# Autodesk Inventor assembly: 110033226_iam_04_大橋塔樓
(part 2 of 2)
981. 110033226_ipt_10_木板條:51
982. 110033226_ipt_10_木板條:52
983. 110033226_ipt_10_木板條:53
984. 110033226_ipt_10_木板條:54
985. 110033226_ipt_10_木板條:55
986. 110033226_ipt_10_木板條:56
987. 110033226_ipt_10_木板條:57
988. 110033226_ipt_10_木板條:58
989. 110033226_ipt_10_木板條:59
990. 110033226_ipt_10_木板條:60
991. 110033226_ipt_10_木板條:61
992. 110033226_ipt_10_木板條:62
993. 110033226_ipt_10_木板條:63
994. 110033226_ipt_10_木板條:64
995. 110033226_ipt_10_木板條:65
996. 110033226_ipt_10_木板條:66
997. 110033226_ipt_10_木板條:67
998. 110033226_ipt_10_木板條:68
999. 110033226_ipt_10_木板條:69
1000. 110033226_ipt_10_木板條:70
1001. 110033226_ipt_10_木板條:71
1002. 110033226_ipt_10_木板條:72
1003. 110033226_ipt_10_木板條:73
1004. 110033226_ipt_10_木板條:74
1005. 110033226_ipt_10_木板條:75
1006. 110033226_ipt_22_塔樓牆壁:238 — 貼合:219, 貼合:220, 貼合:221
1007. 110033226_ipt_22_塔樓牆壁:241
1008. 110033226_ipt_22_塔樓牆壁:242
1009. 110033226_ipt_22_塔樓牆壁:243
1010. 110033226_ipt_22_塔樓牆壁:236 — 貼合:222, 貼合:223, 貼合:224
1011. 110033226_ipt_22_塔樓牆壁:244
1012. 110033226_ipt_22_塔樓牆壁:245
1013. 110033226_ipt_22_塔樓牆壁:240 — 貼合:225, 貼合:226, 貼合:227
1014. 110033226_ipt_22_塔樓牆壁:246
1015. 110033226_ipt_22_塔樓牆壁:247
1016. 110033226_ipt_22_塔樓牆壁:248 — 貼合:228, 貼合:229, 貼合:230
1017. 110033226_ipt_22_塔樓牆壁:249
1018. 110033226_ipt_22_塔樓牆壁:250
1019. 110033226_ipt_22_塔樓牆壁:251
1020. 110033226_ipt_22_塔樓牆壁:252
1021. 110033226_ipt_22_塔樓牆壁:253
1022. 110033226_ipt_22_塔樓牆壁:254
1023. 110033226_ipt_22_塔樓牆壁:255
1024. 110033226_ipt_22_塔樓牆壁:256
1025. 110033226_ipt_22_塔樓牆壁:257
1026. 110033226_ipt_22_塔樓牆壁:258
1027. 110033226_ipt_22_塔樓牆壁:259
1028. 110033226_ipt_22_塔樓牆壁:260
1029. 110033226_ipt_22_塔樓牆壁:261 — 貼合:239
1030. 110033226_ipt_22_塔樓牆壁:262
1031. 110033226_ipt_22_塔樓牆壁:263
1032. 110033226_ipt_22_塔樓牆壁:264
1033. 110033226_ipt_22_塔樓牆壁:265
1034. 110033226_ipt_22_塔樓牆壁:266
1035. 110033226_ipt_22_塔樓牆壁:267
1036. 110033226_ipt_22_塔樓牆壁:268
1037. 110033226_ipt_22_塔樓牆壁:269
1038. 110033226_ipt_22_塔樓牆壁:270
1039. 110033226_ipt_22_塔樓牆壁:271
1040. 110033226_ipt_22_塔樓牆壁:272
1041. 110033226_ipt_22_塔樓牆壁:273 — 貼合:237, 貼合:238
1042. 110033226_ipt_22_塔樓牆壁:274
1043. 110033226_ipt_22_塔樓牆壁:275
1044. 110033226_ipt_22_塔樓牆壁:276
1045. 110033226_ipt_22_塔樓牆壁:277
1046. 110033226_ipt_22_塔樓牆壁:278
1047. 110033226_ipt_22_塔樓牆壁:279
1048. 110033226_ipt_22_塔樓牆壁:280
1049. 110033226_ipt_22_塔樓牆壁:281
1050. 110033226_ipt_22_塔樓牆壁:282
1051. 110033226_ipt_22_塔樓牆壁:283
1052. 110033226_ipt_22_塔樓牆壁:284
1053. 110033226_ipt_22_塔樓牆壁:285
1054. 110033226_ipt_22_塔樓牆壁:286
1055. 110033226_ipt_22_塔樓牆壁:287
1056. 110033226_ipt_22_塔樓牆壁:288
1057. 110033226_ipt_22_塔樓牆壁:289 — 貼合:234, 貼合:235, 貼合:236
1058. 110033226_ipt_22_塔樓牆壁:290
1059. 110033226_ipt_22_塔樓牆壁:291
1060. 110033226_ipt_22_塔樓牆壁:292
1061. 110033226_ipt_22_塔樓牆壁:293
1062. 110033226_ipt_22_塔樓牆壁:294
1063. 110033226_ipt_22_塔樓牆壁:295
1064. 110033226_ipt_22_塔樓牆壁:296
1065. 110033226_ipt_22_塔樓牆壁:297
1066. 110033226_ipt_23_塔樓門口:2 — 貼合:154, 貼合:155, 貼合:156, 貼合:160, 貼合:161, 貼合:162, 貼合:188, 貼合:189
1067. 110033226_ipt_23_塔樓門口:3 — 貼合:187
1068. 110033226_ipt_23_塔樓門口:5
1069. 110033226_ipt_23_塔樓門口:6
1070. 110033226_ipt_23_塔樓門口:7
1071. 110033226_ipt_23_塔樓門口:8
1072. 110033226_ipt_07_磚塊樺木(2x1):229 — 貼合:50, 貼合:51, 貼合:53, 貼合:54, 貼合:56
1073. 110033226_ipt_06_磚塊樺木(1x1):227 — 貼合:54, 貼合:55, 貼合:56
1074. 110033226_ipt_07_磚塊樺木(2x1):230
1075. 110033226_ipt_06_磚塊樺木(1x1):230
1076. 110033226_ipt_07_磚塊樺木(2x1):232 — 貼合:163, 貼合:164
1077. 110033226_ipt_06_磚塊樺木(1x1):232
1078. 110033226_ipt_07_磚塊樺木(2x1):233
1079. 110033226_ipt_06_磚塊樺木(1x1):233 — 貼合:169
1080. 110033226_ipt_07_磚塊樺木(2x1):255
1081. 110033226_ipt_06_磚塊樺木(1x1):255
1082. 110033226_ipt_07_磚塊樺木(2x1):256
1083. 110033226_ipt_06_磚塊樺木(1x1):256
1084. 110033226_ipt_07_磚塊樺木(2x1):257
1085. 110033226_ipt_06_磚塊樺木(1x1):257
1086. 110033226_ipt_07_磚塊樺木(2x1):258
1087. 110033226_ipt_06_磚塊樺木(1x1):258
1088. 110033226_ipt_07_磚塊樺木(2x1):260
1089. 110033226_ipt_06_磚塊樺木(1x1):260
1090. 110033226_ipt_07_磚塊樺木(2x1):261
1091. 110033226_ipt_06_磚塊樺木(1x1):261
1092. 110033226_ipt_07_磚塊樺木(2x1):262
1093. 110033226_ipt_06_磚塊樺木(1x1):262
1094. 110033226_ipt_07_磚塊樺木(2x1):263
1095. 110033226_ipt_06_磚塊樺木(1x1):263
1096. 110033226_ipt_07_磚塊樺木(2x1):265
1097. 110033226_ipt_06_磚塊樺木(1x1):265
1098. 110033226_ipt_07_磚塊樺木(2x1):266
1099. 110033226_ipt_06_磚塊樺木(1x1):266
1100. 110033226_ipt_07_磚塊樺木(2x1):267
1101. 110033226_ipt_06_磚塊樺木(1x1):267
1102. 110033226_ipt_07_磚塊樺木(2x1):268
1103. 110033226_ipt_06_磚塊樺木(1x1):268
1104. 110033226_ipt_07_磚塊樺木(2x1):270
1105. 110033226_ipt_06_磚塊樺木(1x1):270
1106. 110033226_ipt_07_磚塊樺木(2x1):271
1107. 110033226_ipt_06_磚塊樺木(1x1):271
1108. 110033226_ipt_07_磚塊樺木(2x1):272
1109. 110033226_ipt_06_磚塊樺木(1x1):272
1110. 110033226_ipt_07_磚塊樺木(2x1):273
1111. 110033226_ipt_06_磚塊樺木(1x1):273
1112. 110033226_ipt_07_磚塊樺木(2x1):275
1113. 110033226_ipt_06_磚塊樺木(1x1):275
1114. 110033226_ipt_07_磚塊樺木(2x1):276
1115. 110033226_ipt_06_磚塊樺木(1x1):276
1116. 110033226_ipt_07_磚塊樺木(2x1):277
1117. 110033226_ipt_06_磚塊樺木(1x1):277
1118. 110033226_ipt_07_磚塊樺木(2x1):278
1119. 110033226_ipt_06_磚塊樺木(1x1):278
1120. 110033226_ipt_07_磚塊樺木(2x1):280
1121. 110033226_ipt_06_磚塊樺木(1x1):280
1122. 110033226_ipt_07_磚塊樺木(2x1):281
1123. 110033226_ipt_06_磚塊樺木(1x1):281
1124. 110033226_ipt_07_磚塊樺木(2x1):282
1125. 110033226_ipt_06_磚塊樺木(1x1):282
1126. 110033226_ipt_07_磚塊樺木(2x1):283
1127. 110033226_ipt_06_磚塊樺木(1x1):283
1128. 110033226_ipt_07_磚塊樺木(2x1):285
1129. 110033226_ipt_06_磚塊樺木(1x1):285
1130. 110033226_ipt_07_磚塊樺木(2x1):286
1131. 110033226_ipt_06_磚塊樺木(1x1):286
1132. 110033226_ipt_07_磚塊樺木(2x1):287
1133. 110033226_ipt_06_磚塊樺木(1x1):287
1134. 110033226_ipt_07_磚塊樺木(2x1):288
1135. 110033226_ipt_06_磚塊樺木(1x1):288
1136. 110033226_ipt_07_磚塊樺木(2x1):290
1137. 110033226_ipt_06_磚塊樺木(1x1):290
1138. 110033226_ipt_07_磚塊樺木(2x1):291
1139. 110033226_ipt_06_磚塊樺木(1x1):291
1140. 110033226_ipt_07_磚塊樺木(2x1):292
1141. 110033226_ipt_06_磚塊樺木(1x1):292
1142. 110033226_ipt_07_磚塊樺木(2x1):293
1143. 110033226_ipt_06_磚塊樺木(1x1):293
1144. 110033226_ipt_07_磚塊樺木(2x1):295
1145. 110033226_ipt_06_磚塊樺木(1x1):295
1146. 110033226_ipt_07_磚塊樺木(2x1):296
1147. 110033226_ipt_06_磚塊樺木(1x1):296
1148. 110033226_ipt_07_磚塊樺木(2x1):297
1149. 110033226_ipt_06_磚塊樺木(1x1):297
1150. 110033226_ipt_07_磚塊樺木(2x1):298 — 貼合:240
1151. 110033226_ipt_06_磚塊樺木(1x1):298
## Component patterns: (2 elements), (2 elements), (2 elements, first: 110033226_ipt_16_圍牆:1), (12 elements), (2 elements), (14 elements, first: 110033226_ipt_21_柵欄:1), (10 elements, first: 110033226_ipt_21_柵欄:2), (4 elements), (3 elements), (25 elements, first: 110033226_ipt_22_塔樓牆壁:2), (10 elements, first: 110033226_ipt_22_塔樓牆壁:46), (6 elements, first: 110033226_ipt_11_樓梯支架:41), (3 elements, first: 110033226_ipt_10_木板條:3), (6 elements, first: 110033226_ipt_11_樓梯支架:40), (2 elements, first: 110033226_ipt_10_木板條:39), (3 elements), (7 elements, first: 110033226_ipt_22_塔樓牆壁:55), (2 elements, first: 110033226_ipt_22_塔樓牆壁:147), (14 elements, first: 110033226_ipt_22_塔樓牆壁:148), (5 elements), (2 elements), (20 elements, first: 110033226_ipt_07_磚塊樺木(2x1):234 + 110033226_ipt_06_磚塊樺木(1x1):234), (10 elements, first: 110033226_ipt_07_磚塊樺木(2x1):228 + 110033226_ipt_06_磚塊樺木(1x1):229), (10 elements, first: 110033226_ipt_06_磚塊樺木(1x1):299), (4 elements, first: 110033226_ipt_24_直條(3x1):1), (5 elements, first: 110033226_ipt_22_塔樓牆壁:194), (3 elements, first: 110033226_ipt_24_直條(3x1):5), (2 elements), (6 elements, first: 110033226_ipt_22_塔樓牆壁:193), (8 elements, first: 110033226_ipt_22_塔樓牆壁:217), (2 elements, first: 110033226_ipt_22_塔樓牆壁:225), (14 elements, first: 110033226_ipt_21_柵欄:26), (30 elements, first: 110033226_ipt_08_平滑面(3x1):67), (8 elements, first: 110033226_ipt_22_塔樓牆壁:227), (2 elements, first: 110033226_ipt_08_平滑面(3x1):100), (6 elements, first: 110033226_ipt_08_平滑面(3x1):101), (2 elements, first: 110033226_ipt_12_平滑面(2x1):1), (12 elements, first: 110033226_ipt_21_柵欄:42), (3 elements, first: 110033226_ipt_18_大橋圍牆:2), (3 elements, first: 110033226_ipt_18_大橋圍牆:1), (5 elements), (28 elements, first: 110033226_ipt_12_平滑面(2x1):4), (3 elements, first: 110033226_ipt_22_塔樓牆壁:298), (3 elements), (14 elements, first: 110033226_ipt_12_平滑面(2x1):35), (4 elements, first: 110033226_ipt_08_平滑面(3x1):110), (12 elements, first: 110033226_ipt_08_平滑面(3x1):108), (28 elements, first: 110033226_ipt_06_磚塊樺木(1x1):2 + 110033226_ipt_07_磚塊樺木(2x1):2 + 110033226_ipt_06_磚塊樺木(1x1):1 + 110033226_ipt_07_磚塊樺木(2x1):5), 元件陣列 2:2 (28 elements), (28 elements, first: 110033226_ipt_07_磚塊樺木(2x1):3 + 110033226_ipt_06_磚塊樺木(1x1):4 + 110033226_ipt_07_磚塊樺木(2x1):6 + 110033226_ipt_06_磚塊樺木(1x1):5), 元件陣列 1:2 (28 elements), (4 elements, first: 110033226_ipt_08_平滑面(3x1):1), 元件陣列 6:2 (4 elements), 元件陣列 6:3 (4 elements), 元件陣列 6:4 (4 elements), 元件陣列 6:5 (4 elements), 元件陣列 6:6 (4 elements), 元件陣列 6:7 (4 elements), 元件陣列 6:8 (4 elements), 元件陣列 6:9 (4 elements), 元件陣列 6:10 (4 elements), 元件陣列 6:11 (4 elements), 元件陣列 6:12 (4 elements), (4 elements, first: 110033226_ipt_08_平滑面(3x1):2), 元件陣列 8:2 (4 elements), (4 elements, first: 110033226_ipt_11_樓梯支架:1 + 110033226_ipt_11_樓梯支架:2), 元件陣列 17:2 (4 elements), 元件陣列 17:3 (4 elements), 元件陣列 17:4 (4 elements), (6 elements, first: 110033226_ipt_22_塔樓牆壁:1), 元件陣列 19:2 (6 elements), 元件陣列 19:3 (6 elements), (12 elements, first: 110033226_ipt_22_塔樓牆壁:104), 元件陣列 29:2 (12 elements), 元件陣列 29:3 (12 elements), (6 elements, first: 110033226_ipt_22_塔樓牆壁:146), 元件陣列 35:2 (6 elements), 元件陣列 35:3 (6 elements), 元件陣列 35:4 (6 elements), 元件陣列 35:5 (6 elements), (6 elements, first: 110033226_ipt_22_塔樓牆壁:192), 元件陣列 37:2 (6 elements), (2 elements), 元件陣列 14:2 (2 elements), 元件陣列 14:3 (2 elements), 元件陣列 14:4 (2 elements), 元件陣列 14:5 (2 elements), 元件陣列 14:6 (2 elements), 元件陣列 14:7 (2 elements), 元件陣列 14:8 (2 elements), 元件陣列 14:9 (2 elements), 元件陣列 14:10 (2 elements), (30 elements, first: 110033226_ipt_10_木板條:2), 元件陣列 23:2 (30 elements), (4 elements, first: 110033226_ipt_22_塔樓牆壁:238), (3 elements, first: 110033226_ipt_22_塔樓牆壁:236), (3 elements, first: 110033226_ipt_22_塔樓牆壁:240), (2 elements, first: 110033226_ipt_22_塔樓牆壁:248), 元件陣列 59:2 (4 elements), 元件陣列 60:2 (3 elements), 元件陣列 61:2 (3 elements), 元件陣列 62:2 (2 elements), 元件陣列 59:3 (4 elements), 元件陣列 60:3 (3 elements), 元件陣列 61:3 (3 elements), 元件陣列 62:3 (2 elements), 元件陣列 59:4 (4 elements), 元件陣列 60:4 (3 elements), 元件陣列 61:4 (3 elements), 元件陣列 62:4 (2 elements), 元件陣列 59:5 (4 elements), 元件陣列 60:5 (3 elements), 元件陣列 61:5 (3 elements), 元件陣列 62:5 (2 elements), (2 elements, first: 110033226_ipt_23_塔樓門口:2), 元件陣列 34:2 (2 elements), 元件陣列 34:3 (2 elements), (2 elements, first: 110033226_ipt_07_磚塊樺木(2x1):229 + 110033226_ipt_06_磚塊樺木(1x1):227), 元件陣列 12:2 (2 elements), 元件陣列 12:3 (2 elements), 元件陣列 12:4 (2 elements), 元件陣列 12:5 (2 elements), 元件陣列 12:6 (2 elements), 元件陣列 12:7 (2 elements), 元件陣列 12:8 (2 elements), 元件陣列 12:9 (2 elements), 元件陣列 12:10 (2 elements), 元件陣列 12:11 (2 elements), 元件陣列 12:12 (2 elements), 元件陣列 12:13 (2 elements), 元件陣列 12:14 (2 elements), 元件陣列 12:15 (2 elements), 元件陣列 12:16 (2 elements), 元件陣列 12:17 (2 elements), 元件陣列 12:18 (2 elements), 元件陣列 12:19 (2 elements), 元件陣列 12:20 (2 elements)
## Relationships (245: Mate 241, Symmetry 4)
- 貼合:1 [Mate]: 110033226_ipt_05_房子底座:1 ↔ 110033226_ipt_07_磚塊樺木(2x1):6
- 貼合:2 [Mate]: 110033226_ipt_05_房子底座:1 ↔ 110033226_ipt_07_磚塊樺木(2x1):6
- 貼合:3 [Mate]: 110033226_ipt_05_房子底座:1 ↔ 110033226_ipt_07_磚塊樺木(2x1):6
- 貼合:4 [Mate]: 110033226_ipt_05_房子底座:1 ↔ 110033226_ipt_06_磚塊樺木(1x1):5
- 貼合:5 [Mate]: 110033226_ipt_05_房子底座:1 ↔ 110033226_ipt_06_磚塊樺木(1x1):5
- 貼合:6 [Mate]: 110033226_ipt_07_磚塊樺木(2x1):6 ↔ 110033226_ipt_06_磚塊樺木(1x1):5
- 貼合:7 [Mate]: 110033226_ipt_07_磚塊樺木(2x1):3 ↔ 110033226_ipt_07_磚塊樺木(2x1):6
- 貼合:8 [Mate]: 110033226_ipt_07_磚塊樺木(2x1):3 ↔ 110033226_ipt_07_磚塊樺木(2x1):6
- 貼合:9 [Mate]: 110033226_ipt_07_磚塊樺木(2x1):3 ↔ 110033226_ipt_06_磚塊樺木(1x1):5
- 貼合:10 [Mate]: 110033226_ipt_06_磚塊樺木(1x1):4 ↔ 110033226_ipt_07_磚塊樺木(2x1):6
- 貼合:11 [Mate]: 110033226_ipt_06_磚塊樺木(1x1):4 ↔ 110033226_ipt_07_磚塊樺木(2x1):6
- 貼合:12 [Mate]: 110033226_ipt_07_磚塊樺木(2x1):3 ↔ 110033226_ipt_06_磚塊樺木(1x1):4
- 貼合:13 [Mate]: 110033226_ipt_05_房子底座:1 ↔ 110033226_ipt_07_磚塊樺木(2x1):5
- 貼合:14 [Mate]: 110033226_ipt_05_房子底座:1 ↔ 110033226_ipt_07_磚塊樺木(2x1):5
- 貼合:15 [Mate]: 110033226_ipt_05_房子底座:1 ↔ 110033226_ipt_07_磚塊樺木(2x1):5
- 貼合:16 [Mate]: 110033226_ipt_05_房子底座:1 ↔ 110033226_ipt_06_磚塊樺木(1x1):1
- 貼合:17 [Mate]: 110033226_ipt_05_房子底座:1 ↔ 110033226_ipt_06_磚塊樺木(1x1):1
- 貼合:18 [Mate]: 110033226_ipt_06_磚塊樺木(1x1):1 ↔ 110033226_ipt_07_磚塊樺木(2x1):5
- 貼合:19 [Mate]: 110033226_ipt_07_磚塊樺木(2x1):2 ↔ 110033226_ipt_06_磚塊樺木(1x1):1
- 貼合:20 [Mate]: 110033226_ipt_07_磚塊樺木(2x1):2 ↔ 110033226_ipt_07_磚塊樺木(2x1):5
- 貼合:21 [Mate]: 110033226_ipt_07_磚塊樺木(2x1):2 ↔ 110033226_ipt_06_磚塊樺木(1x1):1
- 貼合:22 [Mate]: 110033226_ipt_06_磚塊樺木(1x1):2 ↔ 110033226_ipt_07_磚塊樺木(2x1):5
- 貼合:23 [Mate]: 110033226_ipt_06_磚塊樺木(1x1):2 ↔ 110033226_ipt_07_磚塊樺木(2x1):2
- 貼合:24 [Mate]: 110033226_ipt_06_磚塊樺木(1x1):2 ↔ 110033226_ipt_07_磚塊樺木(2x1):5
- 貼合:25 [Mate]: 110033226_ipt_16_圍牆:1 ↔ 110033226_ipt_07_磚塊樺木(2x1):172
- 貼合:26 [Mate]: 110033226_ipt_16_圍牆:1 ↔ 110033226_ipt_07_磚塊樺木(2x1):172
- 貼合:27 [Mate]: 110033226_ipt_16_圍牆:1 ↔ 110033226_ipt_07_磚塊樺木(2x1):172
- 貼合:28 [Mate]: 110033226_ipt_07_磚塊樺木(2x1):1 ↔ 110033226_ipt_07_磚塊樺木(2x1):214
- 貼合:29 [Mate]: 110033226_ipt_07_磚塊樺木(2x1):1 ↔ 110033226_ipt_07_磚塊樺木(2x1):214
- 貼合:30 [Mate]: 110033226_ipt_07_磚塊樺木(2x1):1 ↔ 110033226_ipt_06_磚塊樺木(1x1):213
- 貼合:31 [Mate]: 110033226_ipt_07_磚塊樺木(2x1):165 ↔ 110033226_ipt_08_平滑面(3x1):1
- 貼合:32 [Mate]: 110033226_ipt_07_磚塊樺木(2x1):59 ↔ 110033226_ipt_08_平滑面(3x1):1
- 貼合:33 [Mate]: 110033226_ipt_07_磚塊樺木(2x1):163 ↔ 110033226_ipt_08_平滑面(3x1):1
- 貼合:34 [Mate]: 110033226_ipt_07_磚塊樺木(2x1):225 ↔ 110033226_ipt_08_平滑面(3x1):2
- 貼合:35 [Mate]: 110033226_ipt_07_磚塊樺木(2x1):169 ↔ 110033226_ipt_08_平滑面(3x1):2
- 貼合:36 [Mate]: 110033226_ipt_06_磚塊樺木(1x1):224 ↔ 110033226_ipt_08_平滑面(3x1):2
- 貼合:37 [Mate]: 110033226_ipt_20_塔樓窗戶:1 ↔ 110033226_ipt_07_磚塊樺木(2x1):21
- 貼合:38 [Mate]: 110033226_ipt_20_塔樓窗戶:1 ↔ 110033226_ipt_06_磚塊樺木(1x1):50
- 貼合:39 [Mate]: 110033226_ipt_20_塔樓窗戶:1 ↔ 110033226_ipt_07_磚塊樺木(2x1):52
- 貼合:40 [Mate]: 110033226_ipt_20_塔樓窗戶:1 ↔ 110033226_ipt_07_磚塊樺木(2x1):21
- 貼合:41 [Mate]: 110033226_ipt_20_塔樓窗戶:2 ↔ 110033226_ipt_07_磚塊樺木(2x1):201
- 貼合:42 [Mate]: 110033226_ipt_20_塔樓窗戶:2 ↔ 110033226_ipt_06_磚塊樺木(1x1):175
- 貼合:43 [Mate]: 110033226_ipt_20_塔樓窗戶:2 ↔ 110033226_ipt_07_磚塊樺木(2x1):201
- 貼合:44 [Mate]: 110033226_ipt_21_柵欄:1 ↔ 110033226_ipt_08_平滑面(3x1):13
- 貼合:45 [Mate]: 110033226_ipt_21_柵欄:1 ↔ 110033226_ipt_08_平滑面(3x1):13
- 貼合:46 [Mate]: 110033226_ipt_21_柵欄:1 ↔ 110033226_ipt_08_平滑面(3x1):13
- 貼合:47 [Mate]: 110033226_ipt_21_柵欄:2 ↔ 110033226_ipt_08_平滑面(3x1):13
- 貼合:48 [Mate]: 110033226_ipt_21_柵欄:1 ↔ 110033226_ipt_21_柵欄:2
- 貼合:49 [Mate]: 110033226_ipt_21_柵欄:2 ↔ 110033226_ipt_08_平滑面(3x1):12
- 貼合:50 [Mate]: 110033226_ipt_08_平滑面(3x1):48 ↔ 110033226_ipt_07_磚塊樺木(2x1):229
- 貼合:51 [Mate]: 110033226_ipt_08_平滑面(3x1):48 ↔ 110033226_ipt_07_磚塊樺木(2x1):229
- 貼合:53 [Mate]: 110033226_ipt_08_平滑面(3x1):48 ↔ 110033226_ipt_07_磚塊樺木(2x1):229
- 貼合:54 [Mate]: 110033226_ipt_07_磚塊樺木(2x1):229 ↔ 110033226_ipt_06_磚塊樺木(1x1):227
- 貼合:55 [Mate]: 110033226_ipt_08_平滑面(3x1):48 ↔ 110033226_ipt_06_磚塊樺木(1x1):227
- 貼合:56 [Mate]: 110033226_ipt_07_磚塊樺木(2x1):229 ↔ 110033226_ipt_06_磚塊樺木(1x1):227
- 貼合:57 [Mate]: 110033226_ipt_07_磚塊樺木(2x1):228 ↔ 110033226_ipt_08_平滑面(3x1):43
- 貼合:58 [Mate]: 110033226_ipt_07_磚塊樺木(2x1):228 ↔ 110033226_ipt_08_平滑面(3x1):43
- 貼合:59 [Mate]: 110033226_ipt_07_磚塊樺木(2x1):228 ↔ 110033226_ipt_08_平滑面(3x1):39
- 貼合:60 [Mate]: 110033226_ipt_06_磚塊樺木(1x1):229 ↔ 110033226_ipt_08_平滑面(3x1):35
- 貼合:61 [Mate]: 110033226_ipt_07_磚塊樺木(2x1):228 ↔ 110033226_ipt_06_磚塊樺木(1x1):229
- 貼合:62 [Mate]: 110033226_ipt_07_磚塊樺木(2x1):228 ↔ 110033226_ipt_06_磚塊樺木(1x1):229
- 貼合:63 [Mate]: 110033226_ipt_08_平滑面(3x1):37 ↔ 110033226_ipt_11_樓梯支架:1
- 貼合:64 [Mate]: 110033226_ipt_08_平滑面(3x1):37 ↔ 110033226_ipt_11_樓梯支架:1
- 貼合:65 [Mate]: 110033226_ipt_08_平滑面(3x1):41 ↔ 110033226_ipt_11_樓梯支架:1
- 貼合:66 [Mate]: 110033226_ipt_11_樓梯支架:1 ↔ 110033226_ipt_11_樓梯支架:2
- 貼合:67 [Mate]: 110033226_ipt_11_樓梯支架:1 ↔ 110033226_ipt_11_樓梯支架:2
- 貼合:68 [Mate]: 110033226_ipt_11_樓梯支架:1 ↔ 110033226_ipt_11_樓梯支架:2
- 貼合:69 [Mate]: 110033226_ipt_08_平滑面(3x1):58 ↔ 110033226_ipt_11_樓梯支架:27
- 貼合:70 [Mate]: 110033226_ipt_08_平滑面(3x1):58 ↔ 110033226_ipt_11_樓梯支架:19
- 貼合:71 [Mate]: 110033226_ipt_08_平滑面(3x1):58 ↔ 110033226_ipt_11_樓梯支架:27
- 貼合:72 [Mate]: 110033226_ipt_08_平滑面(3x1):59 ↔ 110033226_ipt_11_樓梯支架:35
- 貼合:73 [Mate]: 110033226_ipt_08_平滑面(3x1):59 ↔ 110033226_ipt_11_樓梯支架:27
- 貼合:74 [Mate]: 110033226_ipt_08_平滑面(3x1):59 ↔ 110033226_ipt_11_樓梯支架:19
- 貼合:75 [Mate]: 110033226_ipt_08_平滑面(3x1):60 ↔ 110033226_ipt_11_樓梯支架:10
- 貼合:76 [Mate]: 110033226_ipt_08_平滑面(3x1):61 ↔ 110033226_ipt_11_樓梯支架:33
- 貼合:77 [Mate]: 110033226_ipt_08_平滑面(3x1):64 ↔ 110033226_ipt_11_樓梯支架:7
- 貼合:78 [Mate]: 110033226_ipt_08_平滑面(3x1):62 ↔ 110033226_ipt_11_樓梯支架:8
- 貼合:79 [Mate]: 110033226_ipt_08_平滑面(3x1):65 ↔ 110033226_ipt_11_樓梯支架:6
- 貼合:80 [Mate]: 110033226_ipt_08_平滑面(3x1):63 ↔ 110033226_ipt_11_樓梯支架:20
- 貼合:81 [Mate]: 110033226_ipt_08_平滑面(3x1):66 ↔ 110033226_ipt_11_樓梯支架:2
- 貼合:82 [Mate]: 110033226_ipt_08_平滑面(3x1):60 ↔ 110033226_ipt_11_樓梯支架:10
- 貼合:83 [Mate]: 110033226_ipt_08_平滑面(3x1):60 ↔ 110033226_ipt_11_樓梯支架:18
- 貼合:84 [Mate]: 110033226_ipt_08_平滑面(3x1):61 ↔ 110033226_ipt_11_樓梯支架:17
- 貼合:85 [Mate]: 110033226_ipt_08_平滑面(3x1):61 ↔ 110033226_ipt_11_樓梯支架:9
- 貼合:86 [Mate]: 110033226_ipt_08_平滑面(3x1):62 ↔ 110033226_ipt_11_樓梯支架:16
- 貼合:87 [Mate]: 110033226_ipt_08_平滑面(3x1):62 ↔ 110033226_ipt_11_樓梯支架:16
- 貼合:88 [Mate]: 110033226_ipt_08_平滑面(3x1):64 ↔ 110033226_ipt_11_樓梯支架:23
- 貼合:89 [Mate]: 110033226_ipt_08_平滑面(3x1):64 ↔ 110033226_ipt_11_樓梯支架:23
- 貼合:90 [Mate]: 110033226_ipt_08_平滑面(3x1):65 ↔ 110033226_ipt_11_樓梯支架:22
- 貼合:91 [Mate]: 110033226_ipt_08_平滑面(3x1):65 ↔ 110033226_ipt_11_樓梯支架:22
- 貼合:92 [Mate]: 110033226_ipt_08_平滑面(3x1):66 ↔ 110033226_ipt_11_樓梯支架:21
- 貼合:93 [Mate]: 110033226_ipt_08_平滑面(3x1):66 ↔ 110033226_ipt_11_樓梯支架:21
- 貼合:94 [Mate]: 110033226_ipt_08_平滑面(3x1):63 ↔ 110033226_ipt_11_樓梯支架:12
- 貼合:95 [Mate]: 110033226_ipt_08_平滑面(3x1):63 ↔ 110033226_ipt_11_樓梯支架:12
- 貼合:96 [Mate]: 110033226_ipt_05_房子底座:1 ↔ 110033226_ipt_05_房子底座:2
- 貼合:97 [Mate]: 110033226_ipt_05_房子底座:1 ↔ 110033226_ipt_05_房子底座:2
- 貼合:98 [Mate]: 110033226_ipt_05_房子底座:2 ↔ 110033226_ipt_06_磚塊樺木(1x1):117
- 貼合:99 [Mate]: 110033226_ipt_05_房子底座:2 ↔ 110033226_ipt_22_塔樓牆壁:1
- 貼合:100 [Mate]: 110033226_ipt_05_房子底座:2 ↔ 110033226_ipt_22_塔樓牆壁:1
- 貼合:101 [Mate]: 110033226_ipt_05_房子底座:2 ↔ 110033226_ipt_22_塔樓牆壁:1
- 對稱:1 [Symmetry]: 110033226_ipt_05_房子底座:2 ↔ 110033226_ipt_22_塔樓牆壁:2
- 貼合:102 [Mate]: 110033226_ipt_05_房子底座:2 ↔ 110033226_ipt_22_塔樓牆壁:2
- 貼合:103 [Mate]: 110033226_ipt_05_房子底座:2 ↔ 110033226_ipt_22_塔樓牆壁:2
- 貼合:104 [Mate]: 110033226_ipt_23_塔樓門口:1 ↔ 110033226_ipt_22_塔樓牆壁:17
- 貼合:105 [Mate]: 110033226_ipt_23_塔樓門口:1 ↔ 110033226_ipt_22_塔樓牆壁:16
- 貼合:106 [Mate]: 110033226_ipt_23_塔樓門口:1 ↔ 110033226_ipt_22_塔樓牆壁:19
- 貼合:107 [Mate]: 110033226_ipt_22_塔樓牆壁:46 ↔ 110033226_ipt_22_塔樓牆壁:20
- 貼合:108 [Mate]: 110033226_ipt_22_塔樓牆壁:46 ↔ 110033226_ipt_22_塔樓牆壁:19
- 貼合:109 [Mate]: 110033226_ipt_22_塔樓牆壁:46 ↔ 110033226_ipt_22_塔樓牆壁:20
- 貼合:110 [Mate]: 110033226_ipt_22_塔樓牆壁:16 ↔ 110033226_ipt_10_木板條:2
- 貼合:111 [Mate]: 110033226_ipt_22_塔樓牆壁:16 ↔ 110033226_ipt_10_木板條:2
- 貼合:112 [Mate]: 110033226_ipt_22_塔樓牆壁:16 ↔ 110033226_ipt_10_木板條:2
- 貼合:113 [Mate]: 110033226_ipt_10_木板條:34 ↔ 110033226_ipt_11_樓梯支架:41
- 貼合:114 [Mate]: 110033226_ipt_10_木板條:34 ↔ 110033226_ipt_11_樓梯支架:41
- 貼合:115 [Mate]: 110033226_ipt_10_木板條:34 ↔ 110033226_ipt_10_木板條:30
- 貼合:116 [Mate]: 110033226_ipt_10_木板條:34 ↔ 110033226_ipt_10_木板條:31
- 貼合:117 [Mate]: 110033226_ipt_10_木板條:34 ↔ 110033226_ipt_10_木板條:29
- 貼合:118 [Mate]: 110033226_ipt_10_木板條:34 ↔ 110033226_ipt_11_樓梯支架:41
- 貼合:119 [Mate]: 110033226_ipt_10_木板條:42 ↔ 110033226_ipt_11_樓梯支架:41
- 貼合:120 [Mate]: 110033226_ipt_10_木板條:42 ↔ 110033226_ipt_11_樓梯支架:42
- 貼合:121 [Mate]: 110033226_ipt_10_木板條:42 ↔ 110033226_ipt_11_樓梯支架:41
- 貼合:122 [Mate]: 110033226_ipt_11_樓梯支架:46 ↔ 110033226_ipt_10_木板條:3
- 貼合:123 [Mate]: 110033226_ipt_11_樓梯支架:45 ↔ 110033226_ipt_10_木板條:3
- 貼合:124 [Mate]: 110033226_ipt_11_樓梯支架:46 ↔ 110033226_ipt_10_木板條:3
- 貼合:125 [Mate]: 110033226_ipt_10_木板條:44 ↔ 110033226_ipt_11_樓梯支架:40
- 貼合:126 [Mate]: 110033226_ipt_10_木板條:44 ↔ 110033226_ipt_11_樓梯支架:40
- 貼合:127 [Mate]: 110033226_ipt_10_木板條:44 ↔ 110033226_ipt_11_樓梯支架:40
- 貼合:128 [Mate]: 110033226_ipt_10_木板條:33 ↔ 110033226_ipt_11_樓梯支架:51
- 貼合:129 [Mate]: 110033226_ipt_10_木板條:33 ↔ 110033226_ipt_11_樓梯支架:50
- 貼合:130 [Mate]: 110033226_ipt_10_木板條:33 ↔ 110033226_ipt_11_樓梯支架:51
- 貼合:131 [Mate]: 110033226_ipt_10_木板條:36 ↔ 110033226_ipt_11_樓梯支架:48
- 貼合:132 [Mate]: 110033226_ipt_10_木板條:36 ↔ 110033226_ipt_11_樓梯支架:49
- 貼合:133 [Mate]: 110033226_ipt_10_木板條:36 ↔ 110033226_ipt_11_樓梯支架:48
- 貼合:134 [Mate]: 110033226_ipt_10_木板條:1 ↔ 110033226_ipt_11_樓梯支架:43
- 貼合:135 [Mate]: 110033226_ipt_10_木板條:1 ↔ 110033226_ipt_11_樓梯支架:44
- 貼合:136 [Mate]: 110033226_ipt_10_木板條:1 ↔ 110033226_ipt_11_樓梯支架:44
- 貼合:137 [Mate]: 110033226_ipt_05_房子底座:2 ↔ 110033226_ipt_10_木板條:39
- 貼合:138 [Mate]: 110033226_ipt_05_房子底座:2 ↔ 110033226_ipt_10_木板條:39
- 貼合:139 [Mate]: 110033226_ipt_05_房子底座:2 ↔ 110033226_ipt_10_木板條:39
- 貼合:140 [Mate]: 110033226_ipt_10_木板條:35 ↔ 110033226_ipt_11_樓梯支架:47
- 貼合:141 [Mate]: 110033226_ipt_10_木板條:35 ↔ 110033226_ipt_11_樓梯支架:47
- 貼合:142 [Mate]: 110033226_ipt_10_木板條:35 ↔ 110033226_ipt_11_樓梯支架:40
- 貼合:143 [Mate]: 110033226_ipt_05_房子底座:2 ↔ 110033226_ipt_22_塔樓牆壁:55
- 貼合:144 [Mate]: 110033226_ipt_05_房子底座:2 ↔ 110033226_ipt_22_塔樓牆壁:55
- 貼合:145 [Mate]: 110033226_ipt_05_房子底座:2 ↔ 110033226_ipt_22_塔樓牆壁:55
- 貼合:146 [Mate]: 110033226_ipt_05_房子底座:2 ↔ 110033226_ipt_22_塔樓牆壁:104
- 貼合:147 [Mate]: 110033226_ipt_05_房子底座:2 ↔ 110033226_ipt_22_塔樓牆壁:104
- 貼合:148 [Mate]: 110033226_ipt_07_磚塊樺木(2x1):1 ↔ 110033226_ipt_22_塔樓牆壁:104
- 貼合:149 [Mate]: 110033226_ipt_22_塔樓牆壁:145 ↔ 110033226_ipt_22_塔樓牆壁:147
- 貼合:150 [Mate]: 110033226_ipt_22_塔樓牆壁:145 ↔ 110033226_ipt_22_塔樓牆壁:147
- 貼合:151 [Mate]: 110033226_ipt_22_塔樓牆壁:145 ↔ 110033226_ipt_22_塔樓牆壁:147
- 對稱:2 [Symmetry]: 110033226_ipt_22_塔樓牆壁:55 ↔ 110033226_ipt_22_塔樓牆壁:148
- 貼合:152 [Mate]: 110033226_ipt_22_塔樓牆壁:55 ↔ 110033226_ipt_22_塔樓牆壁:148
- 貼合:153 [Mate]: 110033226_ipt_22_塔樓牆壁:55 ↔ 110033226_ipt_22_塔樓牆壁:148
- 貼合:154 [Mate]: 110033226_ipt_22_塔樓牆壁:129 ↔ 110033226_ipt_23_塔樓門口:2
- 貼合:155 [Mate]: 110033226_ipt_22_塔樓牆壁:129 ↔ 110033226_ipt_23_塔樓門口:2
- 貼合:156 [Mate]: 110033226_ipt_22_塔樓牆壁:135 ↔ 110033226_ipt_23_塔樓門口:2
- 貼合:157 [Mate]: 110033226_ipt_22_塔樓牆壁:135 ↔ 110033226_ipt_22_塔樓牆壁:146
- 貼合:158 [Mate]: 110033226_ipt_22_塔樓牆壁:135 ↔ 110033226_ipt_22_塔樓牆壁:146
- 貼合:159 [Mate]: 110033226_ipt_22_塔樓牆壁:137 ↔ 110033226_ipt_22_塔樓牆壁:146
- 貼合:160 [Mate]: 110033226_ipt_22_塔樓牆壁:192 ↔ 110033226_ipt_23_塔樓門口:2
- 貼合:161 [Mate]: 110033226_ipt_22_塔樓牆壁:192 ↔ 110033226_ipt_23_塔樓門口:2
- 貼合:162 [Mate]: 110033226_ipt_22_塔樓牆壁:192 ↔ 110033226_ipt_23_塔樓門口:2
- 對稱:3 [Symmetry]: 110033226_ipt_07_磚塊樺木(2x1):234 ↔ 110033226_ipt_08_平滑面(3x1):24
- 貼合:163 [Mate]: 110033226_ipt_07_磚塊樺木(2x1):234 ↔ 110033226_ipt_07_磚塊樺木(2x1):232
- 貼合:164 [Mate]: 110033226_ipt_07_磚塊樺木(2x1):234 ↔ 110033226_ipt_07_磚塊樺木(2x1):232
- 貼合:165 [Mate]: 110033226_ipt_07_磚塊樺木(2x1):234 ↔ 110033226_ipt_06_磚塊樺木(1x1):234
- 貼合:166 [Mate]: 110033226_ipt_07_磚塊樺木(2x1):234 ↔ 110033226_ipt_06_磚塊樺木(1x1):234
- 貼合:167 [Mate]: 110033226_ipt_07_磚塊樺木(2x1):234 ↔ 110033226_ipt_06_磚塊樺木(1x1):234
- 對稱:4 [Symmetry]: 110033226_ipt_06_磚塊樺木(1x1):299 ↔ 110033226_ipt_08_平滑面(3x1):23
- 貼合:168 [Mate]: 110033226_ipt_06_磚塊樺木(1x1):299 ↔ 110033226_ipt_08_平滑面(3x1):23
- 貼合:169 [Mate]: 110033226_ipt_06_磚塊樺木(1x1):299 ↔ 110033226_ipt_06_磚塊樺木(1x1):233
- 貼合:170 [Mate]: 110033226_ipt_05_房子底座:2 ↔ 110033226_ipt_24_直條(3x1):1
- 貼合:171 [Mate]: 110033226_ipt_22_塔樓牆壁:41 ↔ 110033226_ipt_24_直條(3x1):1
- 貼合:172 [Mate]: 110033226_ipt_22_塔樓牆壁:41 ↔ 110033226_ipt_24_直條(3x1):1
- 貼合:173 [Mate]: 110033226_ipt_22_塔樓牆壁:45 ↔ 110033226_ipt_22_塔樓牆壁:194
- 貼合:174 [Mate]: 110033226_ipt_22_塔樓牆壁:45 ↔ 110033226_ipt_22_塔樓牆壁:194
- 貼合:175 [Mate]: 110033226_ipt_22_塔樓牆壁:45 ↔ 110033226_ipt_22_塔樓牆壁:194
- 貼合:176 [Mate]: 110033226_ipt_24_直條(3x1):5 ↔ 110033226_ipt_22_塔樓牆壁:21
- 貼合:177 [Mate]: 110033226_ipt_24_直條(3x1):5 ↔ 110033226_ipt_22_塔樓牆壁:21
- 貼合:178 [Mate]: 110033226_ipt_22_塔樓牆壁:151 ↔ 110033226_ipt_24_直條(3x1):5
- 貼合:179 [Mate]: 110033226_ipt_23_塔樓門口:1 ↔ 110033226_ipt_22_塔樓牆壁:193
- 貼合:180 [Mate]: 110033226_ipt_23_塔樓門口:1 ↔ 110033226_ipt_22_塔樓牆壁:193
- 貼合:181 [Mate]: 110033226_ipt_23_塔樓門口:1 ↔ 110033226_ipt_22_塔樓牆壁:193
- 貼合:182 [Mate]: 110033226_ipt_23_塔樓門口:1 ↔ 110033226_ipt_24_直條(3x1):8
- 貼合:183 [Mate]: 110033226_ipt_23_塔樓門口:1 ↔ 110033226_ipt_24_直條(3x1):8
- 貼合:184 [Mate]: 110033226_ipt_22_塔樓牆壁:208 ↔ 110033226_ipt_22_塔樓牆壁:217
- 貼合:185 [Mate]: 110033226_ipt_22_塔樓牆壁:209 ↔ 110033226_ipt_22_塔樓牆壁:217
- 貼合:186 [Mate]: 110033226_ipt_22_塔樓牆壁:209 ↔ 110033226_ipt_22_塔樓牆壁:217
- 貼合:187 [Mate]: 110033226_ipt_22_塔樓牆壁:225 ↔ 110033226_ipt_23_塔樓門口:3
- 貼合:188 [Mate]: 110033226_ipt_22_塔樓牆壁:225 ↔ 110033226_ipt_23_塔樓門口:2
- 貼合:189 [Mate]: 110033226_ipt_22_塔樓牆壁:225 ↔ 110033226_ipt_23_塔樓門口:2
- 貼合:190 [Mate]: 110033226_ipt_22_塔樓牆壁:226 ↔ 110033226_ipt_21_柵欄:26
- 貼合:191 [Mate]: 110033226_ipt_22_塔樓牆壁:226 ↔ 110033226_ipt_21_柵欄:26
- 貼合:192 [Mate]: 110033226_ipt_22_塔樓牆壁:226 ↔ 110033226_ipt_21_柵欄:26
- 貼合:193 [Mate]: 110033226_ipt_08_平滑面(3x1):58 ↔ 110033226_ipt_08_平滑面(3x1):67
- 貼合:194 [Mate]: 110033226_ipt_08_平滑面(3x1):58 ↔ 110033226_ipt_08_平滑面(3x1):67
- 貼合:195 [Mate]: 110033226_ipt_08_平滑面(3x1):58 ↔ 110033226_ipt_08_平滑面(3x1):67
- 貼合:196 [Mate]: 110033226_ipt_25_塔樓大窗戶:1 ↔ 110033226_ipt_22_塔樓牆壁:142
- 貼合:197 [Mate]: 110033226_ipt_25_塔樓大窗戶:1 ↔ 110033226_ipt_22_塔樓牆壁:158
- 貼合:198 [Mate]: 110033226_ipt_25_塔樓大窗戶:1 ↔ 110033226_ipt_22_塔樓牆壁:147
- 貼合:199 [Mate]: 110033226_ipt_22_塔樓牆壁:161 ↔ 110033226_ipt_22_塔樓牆壁:227
- 貼合:200 [Mate]: 110033226_ipt_22_塔樓牆壁:161 ↔ 110033226_ipt_22_塔樓牆壁:227
- 貼合:201 [Mate]: 110033226_ipt_22_塔樓牆壁:161 ↔ 110033226_ipt_22_塔樓牆壁:227
- 貼合:202 [Mate]: 110033226_ipt_08_平滑面(3x1):58 ↔ 110033226_ipt_08_平滑面(3x1):100
- 貼合:203 [Mate]: 110033226_ipt_08_平滑面(3x1):70 ↔ 110033226_ipt_08_平滑面(3x1):100
- 貼合:204 [Mate]: 110033226_ipt_08_平滑面(3x1):58 ↔ 110033226_ipt_08_平滑面(3x1):100
- 貼合:205 [Mate]: 110033226_ipt_22_塔樓牆壁:162 ↔ 110033226_ipt_08_平滑面(3x1):101
- 貼合:206 [Mate]: 110033226_ipt_08_平滑面(3x1):95 ↔ 110033226_ipt_08_平滑面(3x1):101
- 貼合:207 [Mate]: 110033226_ipt_08_平滑面(3x1):98 ↔ 110033226_ipt_08_平滑面(3x1):101
- 貼合:208 [Mate]: 110033226_ipt_08_平滑面(3x1):71 ↔ 110033226_ipt_12_平滑面(2x1):1
- 貼合:209 [Mate]: 110033226_ipt_08_平滑面(3x1):104 ↔ 110033226_ipt_12_平滑面(2x1):1
- 貼合:210 [Mate]: 110033226_ipt_08_平滑面(3x1):102 ↔ 110033226_ipt_12_平滑面(2x1):1
- 貼合:211 [Mate]: 110033226_ipt_22_塔樓牆壁:235 ↔ 110033226_ipt_21_柵欄:42
- 貼合:212 [Mate]: 110033226_ipt_22_塔樓牆壁:235 ↔ 110033226_ipt_21_柵欄:42
- 貼合:213 [Mate]: 110033226_ipt_22_塔樓牆壁:216 ↔ 110033226_ipt_18_大橋圍牆:2
- 貼合:214 [Mate]: 110033226_ipt_22_塔樓牆壁:216 ↔ 110033226_ipt_18_大橋圍牆:2
- 貼合:215 [Mate]: 110033226_ipt_22_塔樓牆壁:51 ↔ 110033226_ipt_18_大橋圍牆:2
- 貼合:216 [Mate]: 110033226_ipt_22_塔樓牆壁:224 ↔ 110033226_ipt_18_大橋圍牆:1
- 貼合:217 [Mate]: 110033226_ipt_22_塔樓牆壁:224 ↔ 110033226_ipt_18_大橋圍牆:1
- 貼合:218 [Mate]: 110033226_ipt_22_塔樓牆壁:222 ↔ 110033226_ipt_18_大橋圍牆:1
- 貼合:219 [Mate]: 110033226_ipt_12_平滑面(2x1):1 ↔ 110033226_ipt_22_塔樓牆壁:238
- 貼合:220 [Mate]: 110033226_ipt_08_平滑面(3x1):104 ↔ 110033226_ipt_22_塔樓牆壁:238
- 貼合:221 [Mate]: 110033226_ipt_12_平滑面(2x1):1 ↔ 110033226_ipt_22_塔樓牆壁:238
- 貼合:222 [Mate]: 110033226_ipt_08_平滑面(3x1):71 ↔ 110033226_ipt_22_塔樓牆壁:236
- 貼合:223 [Mate]: 110033226_ipt_08_平滑面(3x1):71 ↔ 110033226_ipt_22_塔樓牆壁:236
- 貼合:224 [Mate]: 110033226_ipt_08_平滑面(3x1):71 ↔ 110033226_ipt_22_塔樓牆壁:236
- 貼合:225 [Mate]: 110033226_ipt_08_平滑面(3x1):73 ↔ 110033226_ipt_22_塔樓牆壁:240
- 貼合:226 [Mate]: 110033226_ipt_08_平滑面(3x1):73 ↔ 110033226_ipt_22_塔樓牆壁:240
- 貼合:227 [Mate]: 110033226_ipt_08_平滑面(3x1):76 ↔ 110033226_ipt_22_塔樓牆壁:240
- 貼合:228 [Mate]: 110033226_ipt_08_平滑面(3x1):91 ↔ 110033226_ipt_22_塔樓牆壁:248
- 貼合:229 [Mate]: 110033226_ipt_08_平滑面(3x1):91 ↔ 110033226_ipt_22_塔樓牆壁:248
- 貼合:230 [Mate]: 110033226_ipt_08_平滑面(3x1):91 ↔ 110033226_ipt_22_塔樓牆壁:248
- 貼合:234 [Mate]: 110033226_ipt_12_平滑面(2x1):4 ↔ 110033226_ipt_22_塔樓牆壁:289
- 貼合:235 [Mate]: 110033226_ipt_12_平滑面(2x1):4 ↔ 110033226_ipt_22_塔樓牆壁:289
- 貼合:236 [Mate]: 110033226_ipt_12_平滑面(2x1):4 ↔ 110033226_ipt_22_塔樓牆壁:289
- 貼合:237 [Mate]: 110033226_ipt_22_塔樓牆壁:298 ↔ 110033226_ipt_22_塔樓牆壁:273
- 貼合:238 [Mate]: 110033226_ipt_22_塔樓牆壁:298 ↔ 110033226_ipt_22_塔樓牆壁:273
- 貼合:239 [Mate]: 110033226_ipt_22_塔樓牆壁:298 ↔ 110033226_ipt_22_塔樓牆壁:261
- 貼合:240 [Mate]: 110033226_ipt_08_平滑面(3x1):110 ↔ 110033226_ipt_07_磚塊樺木(2x1):298
- 貼合:241 [Mate]: 110033226_ipt_06_磚塊樺木(1x1):308 ↔ 110033226_ipt_08_平滑面(3x1):110
- 貼合:242 [Mate]: 110033226_ipt_06_磚塊樺木(1x1):308 ↔ 110033226_ipt_08_平滑面(3x1):110
- 貼合:243 [Mate]: 110033226_ipt_06_磚塊樺木(1x1):308 ↔ 110033226_ipt_08_平滑面(3x1):108
- 貼合:244 [Mate]: 110033226_ipt_06_磚塊樺木(1x1):308 ↔ 110033226_ipt_08_平滑面(3x1):108
- 貼合:245 [Mate]: 110033226_ipt_06_磚塊樺木(1x1):294 ↔ 110033226_ipt_08_平滑面(3x1):108
